# Autodesk Inventor assembly: Assembly_XY_Linear_stage_with_Baseplates_motors_v3
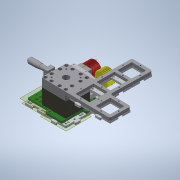
[picture p0: Inventor's stored thumbnail of the model, 180x180]
Saved by Autodesk Inventor 2022 (Build 260153000, 153)
## iProperties
Created: 2021-02-08
Part Number: Assembly_XY_Linear_stage_with_Baseplates_motors_v3
Document SubType Name: Assembly
Designer: diederichbenedict
Author: diederichbenedict
## Documents named in this file (9)
- G:\My Drive\ASP - M.Sc. Photonics\Practical Modules\MODULE 4 - Master Thesis\2.Experiments\Modules\13.XY_Stage_with_Cubes\Assembly_XY_Linear_stage_with_Baseplates_motors_v3.iam
- G:\My Drive\ASP - M.Sc. Photonics\Practical Modules\MODULE 4 - Master Thesis\2.Experiments\Modules\13.XY_Stage_with_Cubes\00_XY_stage-CHUO_SEIKI_LD-647-R1.iam
- G:\My Drive\ASP - M.Sc. Photonics\Practical Modules\MODULE 4 - Master Thesis\2.Experiments\Modules\13.XY_Stage_with_Cubes\30_cellSTORM_UC2_Laser_base.ipt
- G:\My Drive\ASP - M.Sc. Photonics\Practical Modules\MODULE 4 - Master Thesis\2.Experiments\Modules\13.XY_Stage_with_Cubes\30_cellSTORM_UC2_motorized_xystage_spacer.ipt
- G:\My Drive\ASP - M.Sc. Photonics\Practical Modules\MODULE 4 - Master Thesis\2.Experiments\Modules\1.Baseplate\Baseplate_IM\10_Base_puzzle_IM.ipt
- G:\My Drive\ASP - M.Sc. Photonics\Practical Modules\MODULE 4 - Master Thesis\2.Experiments\Modules\13.XY_Stage_with_Cubes\00_micrometer_moun_xystage_china.ipt
- G:\My Drive\ASP - M.Sc. Photonics\Practical Modules\MODULE 4 - Master Thesis\2.Experiments\Modules\13.XY_Stage_with_Cubes\00_micrometer_xy-stage.ipt
- G:\My Drive\ASP - M.Sc. Photonics\Practical Modules\MODULE 4 - Master Thesis\2.Experiments\Modules\13.XY_Stage_with_Cubes\30_XY_Sample_arm_UC2_Adapter_Lighter_v3 - Copy.ipt
- G:\My Drive\ASP - M.Sc. Photonics\Practical Modules\MODULE 4 - Master Thesis\2.Experiments\Modules\13.XY_Stage_with_Cubes\with motor\Assembly_Nema_Motor_attachement_for_XYstage.iam
## Components (17 placed, 8 different names)
1. 00_XY_stage-CHUO_SEIKI_LD-647-R1:1 [sub-assembly] — Rotational:4, Rotational:5, Rotational:6, Rotational:8, Rigid:9
2. 30_cellSTORM_UC2_Laser_base:1 — Mate:1, Mate:2, Flush:1, Mate:3, Rotational:4
3. 30_cellSTORM_UC2_motorized_xystage_spacer:1
4. 10_Base_puzzle_IM:1 — Rigid:2, Flush:3, Rigid:3, Flush:4
5. 10_Base_puzzle_IM:2 — Rigid:3, Flush:4
6. 10_Base_puzzle_IM:3 — Rigid:1, Flush:2
7. 10_Base_puzzle_IM:4 — Mate:1, Mate:2, Flush:1, Mate:3, Rigid:1, Flush:2, Rigid:2, Flush:3
8. 30_XY_Sample_arm_UC2_Adapter_Lighter_v3 - Copy:1 — Rotational:5, Rotational:6, Rotational:7, Rigid:6
9. 00_micrometer_moun_xystage_china:1 — Rotational:2
10. 00_micrometer_moun_xystage_china:2 — Rotational:8, Rotational:9
11. 00_micrometer_xy-stage:1 — Rotational:9
12. 00_micrometer_xy-stage:2 — Rotational:2
13. 10_Base_puzzle_IM:5 — Rigid:7, Rigid:8
14. 10_Base_puzzle_IM:6 — Rigid:5, Rigid:7
15. 10_Base_puzzle_IM:7 — Rigid:5, Rotational:7, Rigid:6
16. 10_Base_puzzle_IM:8 — Rigid:8
17. Assembly_Nema_Motor_attachement_for_XYstage:1 [sub-assembly] — Rigid:9
## Relationships (22: WeldJoint 8, RevoluteJoint 7, Flush 4, Mate 3)
- Mate:1: 30_cellSTORM_UC2_Laser_base:1 ↔ 10_Base_puzzle_IM:4
- Mate:2: 30_cellSTORM_UC2_Laser_base:1 ↔ 10_Base_puzzle_IM:4
- Flush:1: 30_cellSTORM_UC2_Laser_base:1 ↔ 10_Base_puzzle_IM:4
- Mate:3: 30_cellSTORM_UC2_Laser_base:1 ↔ 10_Base_puzzle_IM:4
- Rigid:1 [WeldJoint]: 10_Base_puzzle_IM:3 ↔ 10_Base_puzzle_IM:4
- Flush:2: 10_Base_puzzle_IM:3 ↔ 10_Base_puzzle_IM:4
- Rigid:2 [WeldJoint]: 10_Base_puzzle_IM:1 ↔ 10_Base_puzzle_IM:4
- Flush:3: 10_Base_puzzle_IM:1 ↔ 10_Base_puzzle_IM:4
- Rigid:3 [WeldJoint]: 10_Base_puzzle_IM:1 ↔ 10_Base_puzzle_IM:2
- Flush:4: 10_Base_puzzle_IM:1 ↔ 10_Base_puzzle_IM:2
- Rotational:2 [RevoluteJoint]: 00_micrometer_moun_xystage_china:1 ↔ 00_micrometer_xy-stage:2
- Rigid:5 [WeldJoint]: 10_Base_puzzle_IM:6 ↔ 10_Base_puzzle_IM:7
- Rotational:4 [RevoluteJoint]: 00_XY_stage-CHUO_SEIKI_LD-647-R1:1 ↔ 30_cellSTORM_UC2_Laser_base:1
- Rotational:5 [RevoluteJoint]: 00_XY_stage-CHUO_SEIKI_LD-647-R1:1 ↔ 30_XY_Sample_arm_UC2_Adapter_Lighter_v3 - Copy:1
- Rotational:6 [RevoluteJoint]: 00_XY_stage-CHUO_SEIKI_LD-647-R1:1 ↔ 30_XY_Sample_arm_UC2_Adapter_Lighter_v3 - Copy:1
- Rotational:7 [RevoluteJoint]: 30_XY_Sample_arm_UC2_Adapter_Lighter_v3 - Copy:1 ↔ 10_Base_puzzle_IM:7
- Rigid:6 [WeldJoint]: 30_XY_Sample_arm_UC2_Adapter_Lighter_v3 - Copy:1 ↔ 10_Base_puzzle_IM:7
- Rigid:7 [WeldJoint]: 10_Base_puzzle_IM:5 ↔ 10_Base_puzzle_IM:6
- Rigid:8 [WeldJoint]: 10_Base_puzzle_IM:5 ↔ 10_Base_puzzle_IM:8
- Rotational:8 [RevoluteJoint]: 00_XY_stage-CHUO_SEIKI_LD-647-R1:1 ↔ 00_micrometer_moun_xystage_china:2
- Rotational:9 [RevoluteJoint]: 00_micrometer_moun_xystage_china:2 ↔ 00_micrometer_xy-stage:1
- Rigid:9 [WeldJoint]: 00_XY_stage-CHUO_SEIKI_LD-647-R1:1 ↔ Assembly_Nema_Motor_attachement_for_XYstage:1
